# Autodesk Inventor assembly: Full Assembly
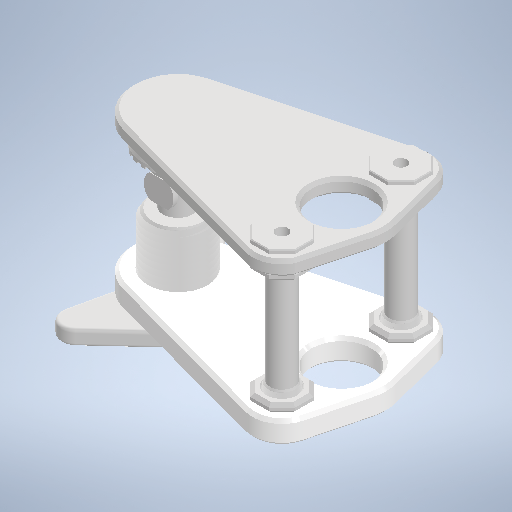
[picture p0: Inventor's stored thumbnail of the model, 512x512]
Saved by Autodesk Inventor 2026.2 (Build 302298010, 298A)
## iProperties
Created: 2026-05-05
Part Number: Full Assembly
Document SubType Name: Assembly
Designer: piete
Author: piete
## Documents named in this file (9)
- C:\Users\piete\Desktop\Skripsie\Documents\Detail Design\Arm Design\Full Assembly.iam
- C:\Users\piete\Desktop\Skripsie\Documents\Detail Design\Arm Design\Bottom Clamp\Bottom Frame.ipt
- C:\Users\piete\Desktop\Skripsie\Documents\Detail Design\Arm Design\Bottom Clamp\Power Screw.ipt
- C:\Users\piete\Desktop\Skripsie\Documents\Detail Design\Arm Design\Bottom Clamp\Foot Stamp.ipt
- C:\Users\piete\Desktop\Skripsie\Documents\Detail Design\Arm Design\Bottom Clamp\Pin.ipt
- C:\Users\piete\Desktop\Skripsie\Documents\Detail Design\Arm Design\Bottom Clamp\Top Frame.ipt
- C:\Users\piete\Desktop\Skripsie\Documents\Detail Design\Arm Design\Bottom Clamp\Small Support.ipt
- C:\Users\piete\Desktop\Skripsie\Documents\Detail Design\Arm Design\Bottom Clamp\Spacer.ipt
- C:\Users\piete\Desktop\Skripsie\Documents\Detail Design\Arm Design\Bottom Clamp\Large Screw.ipt
## Components (13 placed, 8 different names)
1. Bottom Frame:1 — Mate:1, Mate:2, Mate:4, Mate:8, Mate:9, Mate:11, Flush:5, Flush:6, Mate:17, Mate:21
2. Power Screw:1 — Mate:1, Mate:2, Mate:3, Flush:1, Flush:2, Mate:4, Flush:3
3. Foot Stamp:1 — Mate:3, Flush:1, Flush:2, Mate:5, Mate:6, Mate:7
4. Pin:1 — Flush:3, Mate:5, Mate:6
5. Top Frame:1 — Mate:7, Mate:8, Mate:9, Mate:10, Mate:12, Mate:13, Mate:22
6. Small Support:1 — Mate:12, Mate:13, Flush:4, Mate:15, Mate:19, Mate:20
7. Small Support:2 — Mate:10, Mate:11, Flush:4, Mate:14, Mate:16, Mate:18
8. Spacer:1 — Mate:14, Flush:6
9. Spacer:2 — Mate:15, Flush:5
10. Large Screw:1 — Mate:16, Mate:17
11. Large Screw:2 — Mate:18, Flush:7
12. Large Screw:3 — Mate:19, Mate:21
13. Large Screw:4 — Mate:20, Mate:22, Flush:7
## Relationships (29: Mate 22, Flush 7)
- Mate:1: Bottom Frame:1 ↔ Power Screw:1
- Mate:2 (5 mm): Bottom Frame:1 ↔ Power Screw:1
- Mate:3: Power Screw:1 ↔ Foot Stamp:1
- Flush:1: Power Screw:1 ↔ Foot Stamp:1
- Flush:2: Power Screw:1 ↔ Foot Stamp:1
- Mate:4: Bottom Frame:1 ↔ Power Screw:1
- Flush:3 (-10 mm): Power Screw:1 ↔ Pin:1
- Mate:5 (0.2 mm): Foot Stamp:1 ↔ Pin:1
- Mate:6 (0.2 mm): Foot Stamp:1 ↔ Pin:1
- Mate:7: Foot Stamp:1 ↔ Top Frame:1
- Mate:8: Bottom Frame:1 ↔ Top Frame:1
- Mate:9: Bottom Frame:1 ↔ Top Frame:1
- Mate:10: Top Frame:1 ↔ Small Support:2
- Mate:11: Bottom Frame:1 ↔ Small Support:2
- Mate:12: Top Frame:1 ↔ Small Support:1
- Mate:13: Top Frame:1 ↔ Small Support:1
- Flush:4: Small Support:1 ↔ Small Support:2
- Mate:14: Small Support:2 ↔ Spacer:1
- Mate:15: Small Support:1 ↔ Spacer:2
- Flush:5: Bottom Frame:1 ↔ Spacer:2
- Flush:6: Bottom Frame:1 ↔ Spacer:1
- Mate:16: Small Support:2 ↔ Large Screw:1
- Mate:17: Bottom Frame:1 ↔ Large Screw:1
- Mate:18: Small Support:2 ↔ Large Screw:2
- Mate:19: Small Support:1 ↔ Large Screw:3
- Mate:20: Small Support:1 ↔ Large Screw:4
- Mate:21: Bottom Frame:1 ↔ Large Screw:3
- Mate:22: Top Frame:1 ↔ Large Screw:4
- Flush:7: Large Screw:2 ↔ Large Screw:4
